# Autodesk Inventor assembly: ASTRA
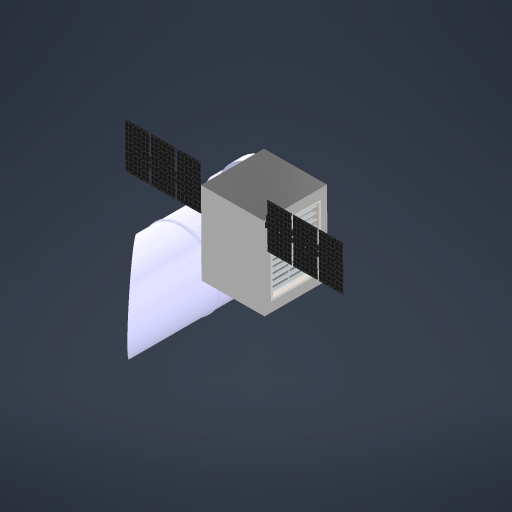
[picture p0: Inventor's stored thumbnail of the model, 512x512]
Saved by Autodesk Inventor 2023.2 (Build 272271030, 271C)
## iProperties
Created: 2023-04-10
Part Number: ASTRA
Document SubType Name: Assembly
Designer: ckeer
Author: ckeer
## Documents named in this file (5)
- F:\Github\School\Prelim\CAD\ASTRA.iam
- F:\Github\School\Prelim\CAD\ASTRA_Body.ipt
- F:\Github\School\Prelim\CAD\automatic-louver-1.snapshot.9\Zip Folder\Louver 061516\Louver 061516\Louver 061516.iam
- F:\Github\School\Prelim\CAD\Sparkwing CAD models 20220411\Sparkwing 1070x570mm 3Panel SA Deployed STEP\Sparkwing 1070x570mm 3Panel SA Deployed STEP.iam
- C:\Users\ckeer\Downloads\OCAMS\OCAMS.ipt
## Components (6 placed, 4 different names)
1. ASTRA_Body:1 — Mate:1, Angle:1, Mate:2, Mate:3, Mate:4, Angle:2, Mate:5, Mate:6
2. Louver 061516:1 [sub-assembly]
3. Louver 061516:2 [sub-assembly]
4. Sparkwing 1070x570mm 3Panel SA Deployed STEP:1 [sub-assembly] — Mate:4, Angle:2, Mate:5, Mate:6
5. Sparkwing 1070x570mm 3Panel SA Deployed STEP:2 [sub-assembly] — Mate:1, Angle:1, Mate:2, Mate:3
6. OCAMS:1
## Relationships (8: Mate 6, Angle 2)
- Mate:1: ASTRA_Body:1 ↔ Sparkwing 1070x570mm 3Panel SA Deployed STEP:2
- Angle:1 (-90 deg): ASTRA_Body:1 ↔ Sparkwing 1070x570mm 3Panel SA Deployed STEP:2
- Mate:2 (-50.8 mm): ASTRA_Body:1 ↔ Sparkwing 1070x570mm 3Panel SA Deployed STEP:2
- Mate:3 (-635 mm): ASTRA_Body:1 ↔ Sparkwing 1070x570mm 3Panel SA Deployed STEP:2
- Mate:4: ASTRA_Body:1 ↔ Sparkwing 1070x570mm 3Panel SA Deployed STEP:1
- Angle:2 (0 deg): ASTRA_Body:1 ↔ Sparkwing 1070x570mm 3Panel SA Deployed STEP:1
- Mate:5 (-50.8 mm): ASTRA_Body:1 ↔ Sparkwing 1070x570mm 3Panel SA Deployed STEP:1
- Mate:6 (-635 mm): ASTRA_Body:1 ↔ Sparkwing 1070x570mm 3Panel SA Deployed STEP:1
